# Autodesk Inventor assembly: Gotowa przekładnia
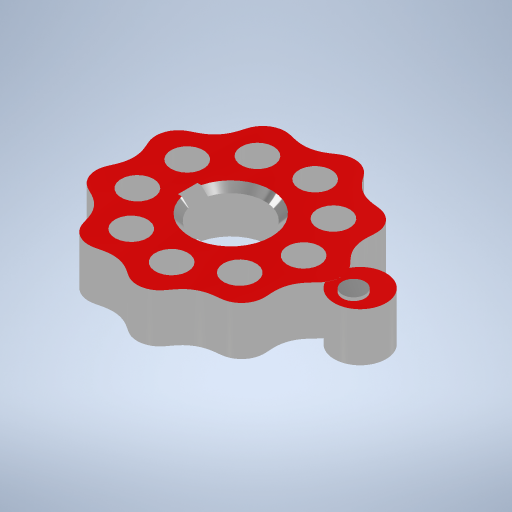
[picture p0: Inventor's stored thumbnail of the model, 512x512]
Saved by Autodesk Inventor 2023 (Build 270158000, 158)
## iProperties
Created: 2023-04-01
Part Number: Gotowa przekładnia
Document SubType Name: Assembly
Designer: Wiktor
Author: Wiktor
## Documents named in this file (3)
- C:\Users\Wiktor\Documents\Manipulator\Gotowa przekładnia.iam
- C:\Users\Wiktor\Documents\Manipulator\Przekładnia cykloidalna mimośrodowa.ipt
- C:\Users\Wiktor\Documents\Manipulator\Przekładnia rolka.ipt
## Components (2 placed, 2 different names)
1. Przekładnia cykloidalna mimośrodowa:1 — Zestawiające:1, Zestawiające:2, Zestawiające:3, Obrót:1
2. Przekładnia rolka:1 — Zestawiające:3, Równoległe:2, Kątowe:1, Obrót:1
## Relationships (6: Mate 3, Flush 1, Angle 1, RelateRotation 1)
- Zestawiające:1 [Mate]: Przekładnia cykloidalna mimośrodowa:1
- Zestawiające:2 [Mate]: Przekładnia cykloidalna mimośrodowa:1
- Zestawiające:3 [Mate] (40 mm): Przekładnia cykloidalna mimośrodowa:1 ↔ Przekładnia rolka:1
- Równoległe:2 [Flush]: Przekładnia rolka:1
- Kątowe:1 [Angle] (0 deg): Przekładnia rolka:1
- Obrót:1 [RelateRotation] (9 ul): Przekładnia cykloidalna mimośrodowa:1 ↔ Przekładnia rolka:1
